# Autodesk Inventor assembly: ProtectionCatapult
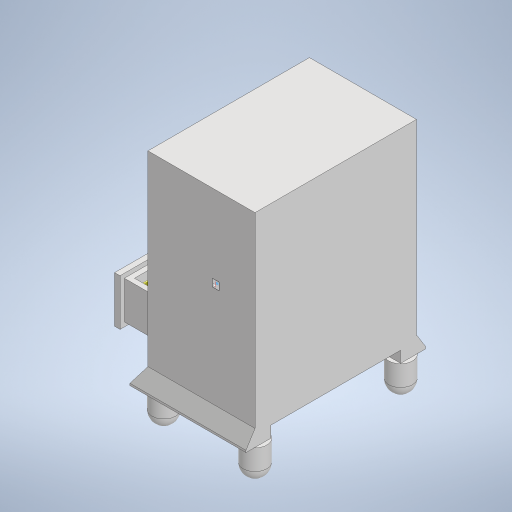
[picture p0: Inventor's stored thumbnail of the model, 512x512]
Saved by Autodesk Inventor 2024 (Build 280153000, 153)
## iProperties
Created: 2025-02-23
Part Number: ProtectionCatapult
Document SubType Name: Assembly
Designer: sergi
Author: sergi
## Documents named in this file (11)
- C:\Users\sergi\OneDrive\Escritorio\GitHub\16. Catapult\Inventor\ProtectionCatapult.iam
- C:\Users\sergi\OneDrive\Escritorio\GitHub\16. Catapult\Inventor\Cajon.ipt
- C:\Users\sergi\OneDrive\Escritorio\GitHub\16. Catapult\Inventor\Comoda.ipt
- C:\Users\sergi\OneDrive\Escritorio\GitHub\16. Catapult\Inventor\NEMA17_Mirror.A.0.ipt
- C:\Users\sergi\OneDrive\Escritorio\GitHub\16. Catapult\Inventor\igus_20250223_174552\103005_para_cremalleras_1\Cremallera103005_para_cremalleras_1.ipt
- C:\Users\sergi\OneDrive\Escritorio\GitHub\16. Catapult\Inventor\igus_20250223_174552\10301_para_engranajes_5\10301_para_engranajes_5.ipt
- C:\Users\sergi\OneDrive\Escritorio\GitHub\16. Catapult\Inventor\Barra deslizante.ipt
- C:\Users\sergi\OneDrive\Escritorio\GitHub\16. Catapult\Inventor\Disco.iam
- C:\Users\sergi\OneDrive\Escritorio\GitHub\16. Catapult\Inventor\Catapulta.iam
- C:\Users\sergi\OneDrive\Escritorio\GitHub\16. Catapult\Inventor\Soporte Motor.ipt
- C:\Users\sergi\OneDrive\Escritorio\GitHub\16. Catapult\Inventor\Soporte Motor Simetrico.ipt
## Components (16 placed, 10 different names)
1. Cajon:1 — Coincidencia:1, Coincidencia:2, Coincidencia:13, Coincidencia:14, Coincidencia:15, Coincidencia:16, Coincidencia:17, Coincidencia:18, Coincidencia:21, Nivelación:9, Coincidencia:23, Nivelación:10, Coincidencia:27, Coincidencia:31
2. Comoda:1 — Coincidencia:1, Coincidencia:2, Coincidencia:3, Coincidencia:4, Coincidencia:5, Coincidencia:6, Coincidencia:7, Coincidencia:8, Coincidencia:9, Coincidencia:10, Coincidencia:11, Coincidencia:12, Nivelación:1, Nivelación:2, Coincidencia:22, Coincidencia:24
3. Cajon:2 — Coincidencia:3, Coincidencia:4, Coincidencia:5
4. Cajon:3 — Coincidencia:6, Coincidencia:7, Coincidencia:8
5. NEMA17_Mirror.A.0:1 — Coincidencia:9, Coincidencia:10, Nivelación:2, Coincidencia:20, Coincidencia:34, Coincidencia:35, Coincidencia:36
6. NEMA17_Mirror.A.0:2 — Coincidencia:11, Coincidencia:12, Nivelación:1, Coincidencia:19, Coincidencia:38, Coincidencia:39, Coincidencia:40
7. Cremallera103005_para_cremalleras_1:1 — Coincidencia:13, Coincidencia:14, Coincidencia:15, Nivelación:8, Rotación/Traslación:1
8. Cremallera103005_para_cremalleras_1:2 — Coincidencia:16, Coincidencia:17, Coincidencia:18, Nivelación:7
9. 10301_para_engranajes_5:1 — Nivelación:7, Coincidencia:20, Rotación:1
10. 10301_para_engranajes_5:2 — Nivelación:8, Coincidencia:19, Rotación/Traslación:1, Rotación:1
11. Barra deslizante:1 — Coincidencia:23, Coincidencia:24, Nivelación:10
12. Barra deslizante:2 — Coincidencia:21, Coincidencia:22, Nivelación:9
13. Catapulta:1 [sub-assembly] — Coincidencia:27, Coincidencia:31, Coincidencia:32, Coincidencia:33, Coincidencia:37
14. Soporte Motor:1 — Coincidencia:38, Coincidencia:39, Coincidencia:40
15. Soporte Motor Simetrico:1 — Coincidencia:34, Coincidencia:35, Coincidencia:36
16. Disco:1 [sub-assembly] — Coincidencia:32, Coincidencia:33, Coincidencia:37
## Relationships (43: Mate 35, Flush 6, RelateRotateTranslate 1, RelateRotation 1)
- Coincidencia:1 [Mate]: Cajon:1 ↔ Comoda:1
- Coincidencia:2 [Mate] (1.5 mm): Cajon:1 ↔ Comoda:1
- Coincidencia:3 [Mate]: Comoda:1 ↔ Cajon:2
- Coincidencia:4 [Mate] (2.5 mm): Comoda:1 ↔ Cajon:2
- Coincidencia:5 [Mate]: Comoda:1 ↔ Cajon:2
- Coincidencia:6 [Mate]: Comoda:1 ↔ Cajon:3
- Coincidencia:7 [Mate]: Comoda:1 ↔ Cajon:3
- Coincidencia:8 [Mate] (2.5 mm): Comoda:1 ↔ Cajon:3
- Coincidencia:9 [Mate]: Comoda:1 ↔ NEMA17_Mirror.A.0:1
- Coincidencia:10 [Mate]: Comoda:1 ↔ NEMA17_Mirror.A.0:1
- Coincidencia:11 [Mate]: Comoda:1 ↔ NEMA17_Mirror.A.0:2
- Coincidencia:12 [Mate]: Comoda:1 ↔ NEMA17_Mirror.A.0:2
- Nivelación:1 [Flush]: Comoda:1 ↔ NEMA17_Mirror.A.0:2
- Nivelación:2 [Flush]: Comoda:1 ↔ NEMA17_Mirror.A.0:1
- Coincidencia:13 [Mate]: Cajon:1 ↔ Cremallera103005_para_cremalleras_1:1
- Coincidencia:14 [Mate]: Cajon:1 ↔ Cremallera103005_para_cremalleras_1:1
- Coincidencia:15 [Mate]: Cajon:1 ↔ Cremallera103005_para_cremalleras_1:1
- Coincidencia:16 [Mate]: Cajon:1 ↔ Cremallera103005_para_cremalleras_1:2
- Coincidencia:17 [Mate]: Cajon:1 ↔ Cremallera103005_para_cremalleras_1:2
- Coincidencia:18 [Mate]: Cajon:1 ↔ Cremallera103005_para_cremalleras_1:2
- Nivelación:7 [Flush]: Cremallera103005_para_cremalleras_1:2 ↔ 10301_para_engranajes_5:1
- Nivelación:8 [Flush]: Cremallera103005_para_cremalleras_1:1 ↔ 10301_para_engranajes_5:2
- Coincidencia:19 [Mate]: NEMA17_Mirror.A.0:2 ↔ 10301_para_engranajes_5:2
- Coincidencia:20 [Mate]: NEMA17_Mirror.A.0:1 ↔ 10301_para_engranajes_5:1
- Coincidencia:21 [Mate]: Cajon:1 ↔ Barra deslizante:2
- Coincidencia:22 [Mate]: Comoda:1 ↔ Barra deslizante:2
- Nivelación:9 [Flush]: Cajon:1 ↔ Barra deslizante:2
- Coincidencia:23 [Mate]: Cajon:1 ↔ Barra deslizante:1
- Coincidencia:24 [Mate]: Comoda:1 ↔ Barra deslizante:1
- Nivelación:10 [Flush]: Cajon:1 ↔ Barra deslizante:1
- Coincidencia:27 [Mate]: Cajon:1 ↔ Catapulta:1
- Coincidencia:31 [Mate]: Cajon:1 ↔ Catapulta:1
- Coincidencia:32 [Mate] (5 mm): Catapulta:1 ↔ Disco:1
- Coincidencia:33 [Mate] (2 mm): Catapulta:1 ↔ Disco:1
- Coincidencia:38 [Mate]: NEMA17_Mirror.A.0:2 ↔ Soporte Motor:1
- Coincidencia:34 [Mate]: NEMA17_Mirror.A.0:1 ↔ Soporte Motor Simetrico:1
- Coincidencia:35 [Mate] (0.2 mm): NEMA17_Mirror.A.0:1 ↔ Soporte Motor Simetrico:1
- Coincidencia:36 [Mate] (0.2 mm): NEMA17_Mirror.A.0:1 ↔ Soporte Motor Simetrico:1
- Coincidencia:37 [Mate] (3 mm): Catapulta:1 ↔ Disco:1
- Coincidencia:39 [Mate] (0.2 mm): NEMA17_Mirror.A.0:2 ↔ Soporte Motor:1
- Coincidencia:40 [Mate] (0.2 mm): NEMA17_Mirror.A.0:2 ↔ Soporte Motor:1
- Rotación/Traslación:1 [RelateRotateTranslate] (16.493 mm): Cremallera103005_para_cremalleras_1:1 ↔ 10301_para_engranajes_5:2
- Rotación:1 [RelateRotation] (1 ul): 10301_para_engranajes_5:1 ↔ 10301_para_engranajes_5:2
